# Autodesk Inventor assembly: Robot_1
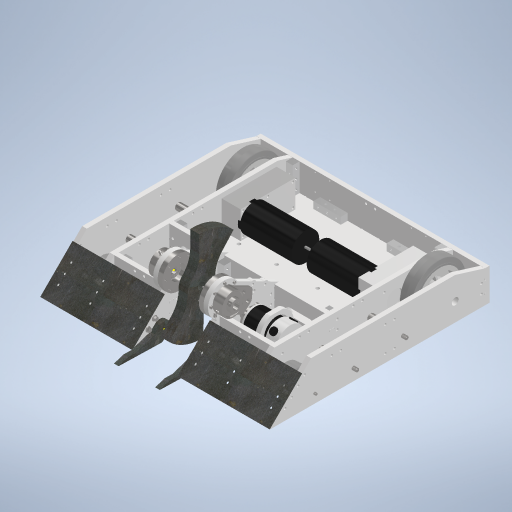
[picture p0: Inventor's stored thumbnail of the model, 512x512]
Saved by Autodesk Inventor 2023 (Build 270158000, 158)
## iProperties
Created: 2023-01-28
Part Number: Robot_1
Document SubType Name: Assembly
Designer: justi
Author: justi
## Documents named in this file (32)
- D:\Final Robot 22-23\Robot_1.iam
- D:\Final Robot 22-23\Base Plate.ipt
- D:\Final Robot 22-23\Side Wall_inner.ipt
- D:\Final Robot 22-23\Components\Block Bracket.ipt
- D:\Final Robot 22-23\Front Wall_inner.ipt
- D:\Final Robot 22-23\Back Wall.ipt
- D:\Final Robot 22-23\Front Wall_outer.ipt
- D:\Final Robot 22-23\Weapon Support Wall_left.ipt
- D:\Final Robot 22-23\Weapon Support Wall_right.ipt
- D:\Final Robot 22-23\Side Wall_outer.ipt
- D:\Final Robot 22-23\Components\0.5in. High-Load Ball Bearing.ipt
- D:\Final Robot 22-23\Weapon Motor Mount_piece1.ipt
- D:\Final Robot 22-23\Motor Mount.ipt
- D:\Final Robot 22-23\Components\A28-150 Motor.ipt
- D:\Final Robot 22-23\Components\0.75in. Ball Bearing.ipt
- D:\Final Robot 22-23\Components\Flanged 0.75in. Mounted Bearing.ipt
- D:\Final Robot 22-23\Components\E30-400 Motor.ipt
- D:\Final Robot 22-23\Components\0.25in. Zinc Yellow-Chromate Plated Hex Head Screw.ipt
- D:\Final Robot 22-23\Components\0.375in. Zinc Yellow-Chromate Plated Hex Head Screw.ipt
- D:\Final Robot 22-23\Components\0.25in. High-Strength Grade 8 Steel Hex Head Screw.ipt
- D:\Final Robot 22-23\Components\0.25in. Grade 8 High-Strength Steel Flange Nut.ipt
- D:\Final Robot 22-23\Components\0.5in. Stainless Steel Unthreaded Spacer.ipt
- D:\Final Robot 22-23\Components\0.375in. Stainless Steel Unthreaded Spacer.ipt
- D:\Final Robot 22-23\Components\6in. x 1.5in. Colson Performa Wheel.ipt
- D:\Final Robot 22-23\Components\3in. x 1.5in. Colson Performa Wheel_BattleKit.ipt
- C:\Users\justi\Documents\test beam.ipt
- D:\Final Robot 22-23\Weapon Hub Support.ipt
- D:\Final Robot 22-23\Components\0.164in. Black-Oxide Alloy Steel Socket Head Screw.ipt
- D:\Final Robot 22-23\Components\0.5in. Wear-Resistant Sprocket-10-Tooth.ipt
- D:\Final Robot 22-23\Wedgelet.ipt
- D:\Final Robot 22-23\Wedge_piece1.ipt
- D:\Final Robot 22-23\Test weapon.ipt
## Components (85 placed, 31 different names)
1. Base Plate:1 — Mate:1, Flush:1, Mate:2, Mate:3, Flush:2, Mate:4, Mate:5, Mate:7, Mate:8, Mate:10, Mate:27, Mate:28, Mate:29, Mate:30, Flush:3, Mate:40, Flush:5, Flush:7, Flush:11, Mate:61, Flush:12, Mate:63, Mate:66, Mate:68, Mate:74, Mate:75, Mate:89, Mate:92
2. Side Wall_inner:1 — Mate:1, Flush:1, Mate:2, Mate:6, Mate:25, Mate:26, Mate:35, Mate:36, Mate:39, Mate:46, Mate:50, Mate:52, Mate:59, Flush:6, Mate:93, Mate:94, Mate:97, Mate:99, Mate:100, Mate:103, Mate:104, Mate:119, Mate:120, Mate:121, Mate:184
3. Side Wall_inner:2 — Mate:3, Flush:2, Mate:4, Mate:9, Mate:23, Mate:24, Mate:37, Mate:38, Flush:4, Mate:43, Mate:47, Mate:48, Mate:49, Mate:51, Mate:60, Flush:8, Flush:9, Mate:90, Mate:91, Mate:95, Mate:101, Mate:102, Mate:105, Mate:106, Mate:122, Mate:123, Mate:124, Mate:186
4. Block Bracket:1 — Mate:8, Mate:9, Mate:10
5. Block Bracket:2 — Mate:23, Mate:24, Mate:49
6. Block Bracket:3 — Mate:25, Mate:26, Mate:50
7. Block Bracket:4 — Mate:53, Mate:54, Mate:55
8. Block Bracket:5 — Mate:5, Mate:6, Mate:7
9. Block Bracket:9 — Mate:27, Mate:28, Mate:65
10. Block Bracket:10 — Mate:29, Mate:30, Mate:64
11. Block Bracket:11 — Mate:37, Mate:38, Mate:51, Mate:96
12. Block Bracket:12 — Mate:35, Mate:36, Mate:52, Mate:98
13. Front Wall_inner:1 — Mate:39, Flush:3, Mate:40, Flush:4, Mate:41, Mate:42, Mate:44, Mate:45, Mate:53, Mate:54, Mate:55, Mate:56, Mate:57, Mate:58, Mate:107, Mate:108, Mate:111, Mate:112
14. Block Bracket:13 — Mate:44, Mate:45, Mate:46
15. Block Bracket:14 — Mate:41, Mate:42, Mate:43, Mate:110
16. Back Wall:1 — Mate:47, Flush:5, Mate:48, Mate:64, Mate:65, Flush:18, Flush:19, Mate:129, Mate:130, Flush:20, Mate:131
17. Block Bracket:15 — Mate:56, Mate:57, Mate:58
18. Front Wall_outer:2 — Mate:60, Flush:8, Flush:9, Mate:62, Mate:67
19. Front Wall_outer:3 — Mate:59, Flush:6, Flush:7, Flush:10, Mate:69
20. Weapon Support Wall_left:1 — Flush:10, Flush:11, Mate:61, Mate:81, Flush:14, Mate:83, Mate:85, Mate:132, Mate:133, Mate:148, Mate:149, Mate:150, Mate:151, Mate:152, Mate:153, Mate:154, Mate:155, Mate:156, Mate:157, Mate:162, Mate:163, Mate:164, Mate:169, Mate:170, Mate:171, Mate:172, Mate:180, Mate:181, Flush:23
21. Weapon Support Wall_right:1 — Mate:62, Flush:12, Mate:63, Mate:70, Flush:13, Mate:72, Mate:73, Mate:82, Flush:15, Mate:86, Mate:88, Mate:135, Mate:137, Mate:138, Mate:139, Mate:140, Mate:141, Mate:142, Mate:143, Mate:144, Mate:145, Mate:146, Mate:147, Mate:159, Mate:160, Mate:161, Mate:165, Mate:166, Mate:167, Mate:168, Mate:182, Mate:183
22. Block Bracket:16 — Mate:68, Mate:69
23. Block Bracket:17 — Mate:66, Mate:67
24. Side Wall_outer:1 — Flush:18, Flush:19, Mate:129, Flush:24
25. Side Wall_outer:2 — Mate:130, Flush:20, Mate:131
26. 0.5in. High-Load Ball Bearing:1 — Mate:70, Flush:13, Mate:71, Mate:77, Mate:78
27. Weapon Motor Mount_piece1:1 — Mate:71, Mate:72, Mate:73, Mate:76, Mate:79, Mate:80
28. Motor Mount:1 — Mate:74, Mate:75
29. 0.5in. High-Load Ball Bearing:2 — Mate:76, Mate:77
30. A28-150 Motor:1 — Mate:78, Mate:79, Mate:80, Mate:158, Flush:21
31. 0.75in. Ball Bearing:1 — Mate:81, Flush:14, Mate:84, Mate:134, Mate:190
32. 0.75in. Ball Bearing:2 — Mate:82, Flush:15, Mate:87, Mate:136
33. Flanged 0.75in. Mounted Bearing:1 — Mate:86, Mate:87, Mate:88
34. Flanged 0.75in. Mounted Bearing:2 — Mate:83, Mate:84, Mate:85
35. E30-400 Motor:1 — Mate:89, Mate:90, Mate:91, Mate:125, Flush:16
36. E30-400 Motor:2 — Mate:92, Mate:93, Mate:94, Mate:126, Flush:17
37. 0.25in. Zinc Yellow-Chromate Plated Hex Head Screw:1 — Mate:95, Mate:96, Mate:115
38. 0.25in. Zinc Yellow-Chromate Plated Hex Head Screw:2 — Mate:97, Mate:98, Mate:116
39. 0.375in. Zinc Yellow-Chromate Plated Hex Head Screw:1 — Mate:103, Mate:104, Mate:117
40. 0.375in. Zinc Yellow-Chromate Plated Hex Head Screw:2 — Mate:99, Mate:100, Mate:118
41. 0.375in. Zinc Yellow-Chromate Plated Hex Head Screw:3 — Mate:101, Mate:102, Mate:114
42. 0.375in. Zinc Yellow-Chromate Plated Hex Head Screw:4 — Mate:105, Mate:106, Mate:113
43. 0.25in. High-Strength Grade 8 Steel Hex Head Screw:1 — Mate:107, Mate:108, Mate:109
44. 0.25in. High-Strength Grade 8 Steel Hex Head Screw:2 — Mate:111, Mate:112
45. 0.25in. Grade 8 High-Strength Steel Flange Nut:1 — Mate:109, Mate:110
46. 0.5in. Stainless Steel Unthreaded Spacer:1 — Mate:115, Mate:124, Mate:128
47. 0.5in. Stainless Steel Unthreaded Spacer:2 — Mate:116, Mate:121, Mate:127
48. 0.375in. Stainless Steel Unthreaded Spacer:1 — Mate:117, Mate:120
49. 0.375in. Stainless Steel Unthreaded Spacer:2 — Mate:113, Mate:123
50. 0.375in. Stainless Steel Unthreaded Spacer:3 — Mate:114, Mate:122
51. 0.375in. Stainless Steel Unthreaded Spacer:4 — Mate:118, Mate:119
52. 6in. x 1.5in. Colson Performa Wheel:1 — Mate:126, Flush:17
53. 6in. x 1.5in. Colson Performa Wheel:2 — Mate:125, Flush:16
54. 3in. x 1.5in. Colson Performa Wheel_BattleKit:1 — Mate:127
55. 3in. x 1.5in. Colson Performa Wheel_BattleKit:2 — Mate:128
56. test beam:1
57. Weapon Hub Support:1 — Mate:135, Mate:136, Mate:137
58. Weapon Hub Support:2 — Mate:132, Mate:133, Mate:134
59. 0.164in. Black-Oxide Alloy Steel Socket Head Screw:1 — Mate:138, Mate:139
60. 0.164in. Black-Oxide Alloy Steel Socket Head Screw:2 — Mate:140, Mate:144
61. 0.164in. Black-Oxide Alloy Steel Socket Head Screw:3 — Mate:141, Mate:145
62. 0.164in. Black-Oxide Alloy Steel Socket Head Screw:4 — Mate:142, Mate:146
63. 0.164in. Black-Oxide Alloy Steel Socket Head Screw:5 — Mate:143, Mate:147
64. 0.164in. Black-Oxide Alloy Steel Socket Head Screw:6 — Mate:148, Mate:157
65. 0.164in. Black-Oxide Alloy Steel Socket Head Screw:7 — Mate:150, Mate:154
66. 0.164in. Black-Oxide Alloy Steel Socket Head Screw:8 — Mate:151, Mate:153
67. 0.164in. Black-Oxide Alloy Steel Socket Head Screw:9 — Mate:152, Mate:155
68. 0.164in. Black-Oxide Alloy Steel Socket Head Screw:10 — Mate:149, Mate:156
69. 0.5in. Wear-Resistant Sprocket-10-Tooth:1 — Mate:158, Flush:21
70. Block Bracket:18 — Mate:159, Mate:160, Mate:161, Mate:178
71. Block Bracket:19 — Mate:162, Mate:163, Mate:164, Mate:174, Mate:176, Mate:185
72. 0.25in. High-Strength Grade 8 Steel Hex Head Screw:3 — Mate:165, Mate:166, Mate:177
73. 0.25in. High-Strength Grade 8 Steel Hex Head Screw:4 — Mate:167, Mate:168, Mate:179
74. 0.25in. High-Strength Grade 8 Steel Hex Head Screw:5 — Mate:169, Mate:171, Mate:173
75. 0.25in. High-Strength Grade 8 Steel Hex Head Screw:6 — Mate:170, Mate:172, Mate:175
76. 0.25in. Grade 8 High-Strength Steel Flange Nut:2 — Mate:177, Mate:178
77. 0.25in. Grade 8 High-Strength Steel Flange Nut:3 — Mate:179
78. 0.25in. Grade 8 High-Strength Steel Flange Nut:4 — Mate:173, Mate:174
79. 0.25in. Grade 8 High-Strength Steel Flange Nut:5 — Mate:175, Mate:176
80. Wedgelet:1 — Mate:180, Mate:181, Flush:22
81. Wedgelet:2 — Mate:182, Mate:183, Flush:22
82. Wedge_piece1:1 — Mate:184, Flush:23, Mate:185, Flush:25
83. Wedge_piece1:2 — Mate:186, Flush:24, Flush:25
84. Test weapon:1 — Mate:187, Mate:188, Mate:189
85. Test weapon:2 — Mate:187, Mate:188, Mate:189, Mate:190
## Relationships (199: Mate 174, Flush 25)
- Mate:1: Base Plate:1 ↔ Side Wall_inner:1
- Flush:1: Base Plate:1 ↔ Side Wall_inner:1
- Mate:2: Base Plate:1 ↔ Side Wall_inner:1
- Mate:3: Base Plate:1 ↔ Side Wall_inner:2
- Flush:2: Base Plate:1 ↔ Side Wall_inner:2
- Mate:4: Base Plate:1 ↔ Side Wall_inner:2
- Mate:5: Base Plate:1 ↔ Block Bracket:5
- Mate:6: Side Wall_inner:1 ↔ Block Bracket:5
- Mate:7: Base Plate:1 ↔ Block Bracket:5
- Mate:8: Base Plate:1 ↔ Block Bracket:1
- Mate:9: Side Wall_inner:2 ↔ Block Bracket:1
- Mate:10: Base Plate:1 ↔ Block Bracket:1
- Mate:23: Side Wall_inner:2 ↔ Block Bracket:2
- Mate:24: Side Wall_inner:2 ↔ Block Bracket:2
- Mate:25: Side Wall_inner:1 ↔ Block Bracket:3
- Mate:26: Side Wall_inner:1 ↔ Block Bracket:3
- Mate:27: Base Plate:1 ↔ Block Bracket:9
- Mate:28: Base Plate:1 ↔ Block Bracket:9
- Mate:29: Base Plate:1 ↔ Block Bracket:10
- Mate:30: Base Plate:1 ↔ Block Bracket:10
- Mate:35: Side Wall_inner:1 ↔ Block Bracket:12
- Mate:36: Side Wall_inner:1 ↔ Block Bracket:12
- Mate:37: Side Wall_inner:2 ↔ Block Bracket:11
- Mate:38: Side Wall_inner:2 ↔ Block Bracket:11
- Mate:39: Side Wall_inner:1 ↔ Front Wall_inner:1
- Flush:3: Base Plate:1 ↔ Front Wall_inner:1
- Mate:40: Base Plate:1 ↔ Front Wall_inner:1
- Flush:4: Side Wall_inner:2 ↔ Front Wall_inner:1
- Mate:41: Front Wall_inner:1 ↔ Block Bracket:14
- Mate:42: Front Wall_inner:1 ↔ Block Bracket:14
- Mate:43: Side Wall_inner:2 ↔ Block Bracket:14
- Mate:44: Front Wall_inner:1 ↔ Block Bracket:13
- Mate:45: Front Wall_inner:1 ↔ Block Bracket:13
- Mate:46: Side Wall_inner:1 ↔ Block Bracket:13
- Mate:47: Side Wall_inner:2 ↔ Back Wall:1
- Flush:5: Base Plate:1 ↔ Back Wall:1
- Mate:48: Side Wall_inner:2 ↔ Back Wall:1
- Mate:49: Side Wall_inner:2 ↔ Block Bracket:2
- Mate:50: Side Wall_inner:1 ↔ Block Bracket:3
- Mate:51: Side Wall_inner:2 ↔ Block Bracket:11
- Mate:52: Side Wall_inner:1 ↔ Block Bracket:12
- Mate:53: Block Bracket:4 ↔ Front Wall_inner:1
- Mate:54: Block Bracket:4 ↔ Front Wall_inner:1
- Mate:55: Block Bracket:4 ↔ Front Wall_inner:1
- Mate:56: Front Wall_inner:1 ↔ Block Bracket:15
- Mate:57: Front Wall_inner:1 ↔ Block Bracket:15
- Mate:58: Front Wall_inner:1 ↔ Block Bracket:15
- Mate:59: Side Wall_inner:1 ↔ Front Wall_outer:3
- Flush:6: Side Wall_inner:1 ↔ Front Wall_outer:3
- Flush:7: Base Plate:1 ↔ Front Wall_outer:3
- Mate:60: Side Wall_inner:2 ↔ Front Wall_outer:2
- Flush:8: Side Wall_inner:2 ↔ Front Wall_outer:2
- Flush:9: Side Wall_inner:2 ↔ Front Wall_outer:2
- Flush:10: Front Wall_outer:3 ↔ Weapon Support Wall_left:1
- Flush:11: Base Plate:1 ↔ Weapon Support Wall_left:1
- Mate:61: Base Plate:1 ↔ Weapon Support Wall_left:1
- Mate:62: Front Wall_outer:2 ↔ Weapon Support Wall_right:1
- Flush:12: Base Plate:1 ↔ Weapon Support Wall_right:1
- Mate:63: Base Plate:1 ↔ Weapon Support Wall_right:1
- Mate:64: Block Bracket:10 ↔ Back Wall:1
- Mate:65: Block Bracket:9 ↔ Back Wall:1
- Mate:66: Base Plate:1 ↔ Block Bracket:17
- Mate:67: Front Wall_outer:2 ↔ Block Bracket:17
- Mate:68: Base Plate:1 ↔ Block Bracket:16
- Mate:69: Front Wall_outer:3 ↔ Block Bracket:16
- Mate:70: Weapon Support Wall_right:1 ↔ 0.5in. High-Load Ball Bearing:1
- Flush:13: Weapon Support Wall_right:1 ↔ 0.5in. High-Load Ball Bearing:1
- Mate:71: 0.5in. High-Load Ball Bearing:1 ↔ Weapon Motor Mount_piece1:1
- Mate:72: Weapon Support Wall_right:1 ↔ Weapon Motor Mount_piece1:1
- Mate:73: Weapon Support Wall_right:1 ↔ Weapon Motor Mount_piece1:1
- Mate:74: Base Plate:1 ↔ Motor Mount:1
- Mate:75: Base Plate:1 ↔ Motor Mount:1
- Mate:76: Weapon Motor Mount_piece1:1 ↔ 0.5in. High-Load Ball Bearing:2
- Mate:77: 0.5in. High-Load Ball Bearing:1 ↔ 0.5in. High-Load Ball Bearing:2
- Mate:78: 0.5in. High-Load Ball Bearing:1 ↔ A28-150 Motor:1
- Mate:79: Weapon Motor Mount_piece1:1 ↔ A28-150 Motor:1
- Mate:80: Weapon Motor Mount_piece1:1 ↔ A28-150 Motor:1
- Mate:81: Weapon Support Wall_left:1 ↔ 0.75in. Ball Bearing:1
- Flush:14: Weapon Support Wall_left:1 ↔ 0.75in. Ball Bearing:1
- Mate:82: Weapon Support Wall_right:1 ↔ 0.75in. Ball Bearing:2
- Flush:15: Weapon Support Wall_right:1 ↔ 0.75in. Ball Bearing:2
- Mate:83: Weapon Support Wall_left:1 ↔ Flanged 0.75in. Mounted Bearing:2
- Mate:84: 0.75in. Ball Bearing:1 ↔ Flanged 0.75in. Mounted Bearing:2
- Mate:85: Weapon Support Wall_left:1 ↔ Flanged 0.75in. Mounted Bearing:2
- Mate:86: Weapon Support Wall_right:1 ↔ Flanged 0.75in. Mounted Bearing:1
- Mate:87: 0.75in. Ball Bearing:2 ↔ Flanged 0.75in. Mounted Bearing:1
- Mate:88: Weapon Support Wall_right:1 ↔ Flanged 0.75in. Mounted Bearing:1
- Mate:89: Base Plate:1 ↔ E30-400 Motor:1
- Mate:90: Side Wall_inner:2 ↔ E30-400 Motor:1
- Mate:91: Side Wall_inner:2 ↔ E30-400 Motor:1
- Mate:92: Base Plate:1 ↔ E30-400 Motor:2
- Mate:93: Side Wall_inner:1 ↔ E30-400 Motor:2
- Mate:94: Side Wall_inner:1 ↔ E30-400 Motor:2
- Mate:95: Side Wall_inner:2 ↔ 0.25in. Zinc Yellow-Chromate Plated Hex Head Screw:1
- Mate:96: Block Bracket:11 ↔ 0.25in. Zinc Yellow-Chromate Plated Hex Head Screw:1
- Mate:97: Side Wall_inner:1 ↔ 0.25in. Zinc Yellow-Chromate Plated Hex Head Screw:2
- Mate:98: Block Bracket:12 ↔ 0.25in. Zinc Yellow-Chromate Plated Hex Head Screw:2
- Mate:99: Side Wall_inner:1 ↔ 0.375in. Zinc Yellow-Chromate Plated Hex Head Screw:2
- Mate:100: Side Wall_inner:1 ↔ 0.375in. Zinc Yellow-Chromate Plated Hex Head Screw:2
- Mate:101: Side Wall_inner:2 ↔ 0.375in. Zinc Yellow-Chromate Plated Hex Head Screw:3
- Mate:102: Side Wall_inner:2 ↔ 0.375in. Zinc Yellow-Chromate Plated Hex Head Screw:3
- Mate:103: Side Wall_inner:1 ↔ 0.375in. Zinc Yellow-Chromate Plated Hex Head Screw:1
- Mate:104: Side Wall_inner:1 ↔ 0.375in. Zinc Yellow-Chromate Plated Hex Head Screw:1
- Mate:105: Side Wall_inner:2 ↔ 0.375in. Zinc Yellow-Chromate Plated Hex Head Screw:4
- Mate:106: Side Wall_inner:2 ↔ 0.375in. Zinc Yellow-Chromate Plated Hex Head Screw:4
- Mate:107: Front Wall_inner:1 ↔ 0.25in. High-Strength Grade 8 Steel Hex Head Screw:1
- Mate:108: Front Wall_inner:1 ↔ 0.25in. High-Strength Grade 8 Steel Hex Head Screw:1
- Mate:109: 0.25in. High-Strength Grade 8 Steel Hex Head Screw:1 ↔ 0.25in. Grade 8 High-Strength Steel Flange Nut:1
- Mate:110: Block Bracket:14 ↔ 0.25in. Grade 8 High-Strength Steel Flange Nut:1
- Mate:111: Front Wall_inner:1 ↔ 0.25in. High-Strength Grade 8 Steel Hex Head Screw:2
- Mate:112: Front Wall_inner:1 ↔ 0.25in. High-Strength Grade 8 Steel Hex Head Screw:2
- Mate:113: 0.375in. Zinc Yellow-Chromate Plated Hex Head Screw:4 ↔ 0.375in. Stainless Steel Unthreaded Spacer:2
- Mate:114: 0.375in. Zinc Yellow-Chromate Plated Hex Head Screw:3 ↔ 0.375in. Stainless Steel Unthreaded Spacer:3
- Mate:115: 0.25in. Zinc Yellow-Chromate Plated Hex Head Screw:1 ↔ 0.5in. Stainless Steel Unthreaded Spacer:1
- Mate:116: 0.25in. Zinc Yellow-Chromate Plated Hex Head Screw:2 ↔ 0.5in. Stainless Steel Unthreaded Spacer:2
- Mate:117: 0.375in. Zinc Yellow-Chromate Plated Hex Head Screw:1 ↔ 0.375in. Stainless Steel Unthreaded Spacer:1
- Mate:118: 0.375in. Zinc Yellow-Chromate Plated Hex Head Screw:2 ↔ 0.375in. Stainless Steel Unthreaded Spacer:4
- Mate:119: Side Wall_inner:1 ↔ 0.375in. Stainless Steel Unthreaded Spacer:4
- Mate:120: Side Wall_inner:1 ↔ 0.375in. Stainless Steel Unthreaded Spacer:1
- Mate:121: Side Wall_inner:1 ↔ 0.5in. Stainless Steel Unthreaded Spacer:2
- Mate:122: Side Wall_inner:2 ↔ 0.375in. Stainless Steel Unthreaded Spacer:3
- Mate:123: Side Wall_inner:2 ↔ 0.375in. Stainless Steel Unthreaded Spacer:2
- Mate:124: Side Wall_inner:2 ↔ 0.5in. Stainless Steel Unthreaded Spacer:1
- Mate:125: E30-400 Motor:1 ↔ 6in. x 1.5in. Colson Performa Wheel:2
- Flush:16: E30-400 Motor:1 ↔ 6in. x 1.5in. Colson Performa Wheel:2
- Mate:126: E30-400 Motor:2 ↔ 6in. x 1.5in. Colson Performa Wheel:1
- Flush:17: E30-400 Motor:2 ↔ 6in. x 1.5in. Colson Performa Wheel:1
- Mate:127: 0.5in. Stainless Steel Unthreaded Spacer:2 ↔ 3in. x 1.5in. Colson Performa Wheel_BattleKit:1
- Mate:128: 0.5in. Stainless Steel Unthreaded Spacer:1 ↔ 3in. x 1.5in. Colson Performa Wheel_BattleKit:2
- Flush:18: Back Wall:1 ↔ Side Wall_outer:1
- Flush:19: Back Wall:1 ↔ Side Wall_outer:1
- Mate:129: Back Wall:1 ↔ Side Wall_outer:1
- Mate:130: Back Wall:1 ↔ Side Wall_outer:2
- Flush:20: Back Wall:1 ↔ Side Wall_outer:2
- Mate:131: Back Wall:1 ↔ Side Wall_outer:2
- Mate:132: Weapon Support Wall_left:1 ↔ Weapon Hub Support:2
- Mate:133: Weapon Support Wall_left:1 ↔ Weapon Hub Support:2
- Mate:134: 0.75in. Ball Bearing:1 ↔ Weapon Hub Support:2
- Mate:135: Weapon Support Wall_right:1 ↔ Weapon Hub Support:1
- Mate:136: 0.75in. Ball Bearing:2 ↔ Weapon Hub Support:1
- Mate:137: Weapon Support Wall_right:1 ↔ Weapon Hub Support:1
- Mate:138: Weapon Support Wall_right:1 ↔ 0.164in. Black-Oxide Alloy Steel Socket Head Screw:1
- Mate:139: Weapon Support Wall_right:1 ↔ 0.164in. Black-Oxide Alloy Steel Socket Head Screw:1
- Mate:140: Weapon Support Wall_right:1 ↔ 0.164in. Black-Oxide Alloy Steel Socket Head Screw:2
- Mate:141: Weapon Support Wall_right:1 ↔ 0.164in. Black-Oxide Alloy Steel Socket Head Screw:3
- Mate:142: Weapon Support Wall_right:1 ↔ 0.164in. Black-Oxide Alloy Steel Socket Head Screw:4
- Mate:143: Weapon Support Wall_right:1 ↔ 0.164in. Black-Oxide Alloy Steel Socket Head Screw:5
- Mate:144: Weapon Support Wall_right:1 ↔ 0.164in. Black-Oxide Alloy Steel Socket Head Screw:2
- Mate:145: Weapon Support Wall_right:1 ↔ 0.164in. Black-Oxide Alloy Steel Socket Head Screw:3
- Mate:146: Weapon Support Wall_right:1 ↔ 0.164in. Black-Oxide Alloy Steel Socket Head Screw:4
- Mate:147: Weapon Support Wall_right:1 ↔ 0.164in. Black-Oxide Alloy Steel Socket Head Screw:5
- Mate:148: Weapon Support Wall_left:1 ↔ 0.164in. Black-Oxide Alloy Steel Socket Head Screw:6
- Mate:149: Weapon Support Wall_left:1 ↔ 0.164in. Black-Oxide Alloy Steel Socket Head Screw:10
- Mate:150: Weapon Support Wall_left:1 ↔ 0.164in. Black-Oxide Alloy Steel Socket Head Screw:7
- Mate:151: Weapon Support Wall_left:1 ↔ 0.164in. Black-Oxide Alloy Steel Socket Head Screw:8
- Mate:152: Weapon Support Wall_left:1 ↔ 0.164in. Black-Oxide Alloy Steel Socket Head Screw:9
- Mate:153: Weapon Support Wall_left:1 ↔ 0.164in. Black-Oxide Alloy Steel Socket Head Screw:8
- Mate:154: Weapon Support Wall_left:1 ↔ 0.164in. Black-Oxide Alloy Steel Socket Head Screw:7
- Mate:155: Weapon Support Wall_left:1 ↔ 0.164in. Black-Oxide Alloy Steel Socket Head Screw:9
- Mate:156: Weapon Support Wall_left:1 ↔ 0.164in. Black-Oxide Alloy Steel Socket Head Screw:10
- Mate:157: Weapon Support Wall_left:1 ↔ 0.164in. Black-Oxide Alloy Steel Socket Head Screw:6
- Mate:158: A28-150 Motor:1 ↔ 0.5in. Wear-Resistant Sprocket-10-Tooth:1
- Flush:21: A28-150 Motor:1 ↔ 0.5in. Wear-Resistant Sprocket-10-Tooth:1
- Mate:159: Weapon Support Wall_right:1 ↔ Block Bracket:18
- Mate:160: Weapon Support Wall_right:1 ↔ Block Bracket:18
- Mate:161: Weapon Support Wall_right:1 ↔ Block Bracket:18
- Mate:162: Weapon Support Wall_left:1 ↔ Block Bracket:19
- Mate:163: Weapon Support Wall_left:1 ↔ Block Bracket:19
- Mate:164: Weapon Support Wall_left:1 ↔ Block Bracket:19
- Mate:165: Weapon Support Wall_right:1 ↔ 0.25in. High-Strength Grade 8 Steel Hex Head Screw:3
- Mate:166: Weapon Support Wall_right:1 ↔ 0.25in. High-Strength Grade 8 Steel Hex Head Screw:3
- Mate:167: Weapon Support Wall_right:1 ↔ 0.25in. High-Strength Grade 8 Steel Hex Head Screw:4
- Mate:168: Weapon Support Wall_right:1 ↔ 0.25in. High-Strength Grade 8 Steel Hex Head Screw:4
- Mate:169: Weapon Support Wall_left:1 ↔ 0.25in. High-Strength Grade 8 Steel Hex Head Screw:5
- Mate:170: Weapon Support Wall_left:1 ↔ 0.25in. High-Strength Grade 8 Steel Hex Head Screw:6
- Mate:171: Weapon Support Wall_left:1 ↔ 0.25in. High-Strength Grade 8 Steel Hex Head Screw:5
- Mate:172: Weapon Support Wall_left:1 ↔ 0.25in. High-Strength Grade 8 Steel Hex Head Screw:6
- Mate:173: 0.25in. High-Strength Grade 8 Steel Hex Head Screw:5 ↔ 0.25in. Grade 8 High-Strength Steel Flange Nut:4
- Mate:174: Block Bracket:19 ↔ 0.25in. Grade 8 High-Strength Steel Flange Nut:4
- Mate:175: 0.25in. High-Strength Grade 8 Steel Hex Head Screw:6 ↔ 0.25in. Grade 8 High-Strength Steel Flange Nut:5
- Mate:176: Block Bracket:19 ↔ 0.25in. Grade 8 High-Strength Steel Flange Nut:5
- Mate:177: 0.25in. High-Strength Grade 8 Steel Hex Head Screw:3 ↔ 0.25in. Grade 8 High-Strength Steel Flange Nut:2
- Mate:178: Block Bracket:18 ↔ 0.25in. Grade 8 High-Strength Steel Flange Nut:2
- Mate:179: 0.25in. High-Strength Grade 8 Steel Hex Head Screw:4 ↔ 0.25in. Grade 8 High-Strength Steel Flange Nut:3
- Mate:180: Weapon Support Wall_left:1 ↔ Wedgelet:1
- Mate:181: Weapon Support Wall_left:1 ↔ Wedgelet:1
- Mate:182: Weapon Support Wall_right:1 ↔ Wedgelet:2
- Mate:183: Weapon Support Wall_right:1 ↔ Wedgelet:2
- Flush:22: Wedgelet:1 ↔ Wedgelet:2
- Mate:184: Side Wall_inner:1 ↔ Wedge_piece1:1
- Flush:23: Weapon Support Wall_left:1 ↔ Wedge_piece1:1
- Mate:185: Block Bracket:19 ↔ Wedge_piece1:1
- Mate:186: Side Wall_inner:2 ↔ Wedge_piece1:2
- Flush:24: Side Wall_outer:1 ↔ Wedge_piece1:2
- Flush:25: Wedge_piece1:1 ↔ Wedge_piece1:2
- Mate:187: Test weapon:1 ↔ Test weapon:2
- Mate:188: Test weapon:1 ↔ Test weapon:2
- Mate:189: Test weapon:1 ↔ Test weapon:2
- Mate:190: 0.75in. Ball Bearing:1 ↔ Test weapon:2
